# Autodesk Inventor assembly: bett_V3_teil3_klappe
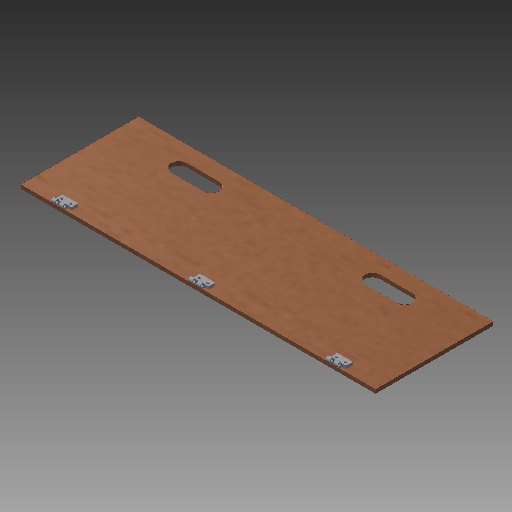
[picture p0: Inventor's stored thumbnail of the model, 512x512]
Saved by Autodesk Inventor 2018 (Build 220112000, 112)
## iProperties
Created: 2020-03-29
Part Number: bett_V3_teil3_klappe
Material: Generisch
Document SubType Name: Assembly
Designer: wepet
Mass: 2.61491 g
Surface Area: 84.4948 cm^2
Volume: 4.7078 cm^3
Density: 0.555441 g/cm^3
Author: wepet
## Documents named in this file (4)
- C:\Users\wepet\Downloads\anhaenger\current\details\bett\bett_V3\bett_V3_teil3_klappe.iam
- C:\Users\wepet\Downloads\anhaenger\current\details\bett\bett_V3\bett_V3_detail_deckplatte_klappe.ipt
- C:\Users\wepet\Downloads\anhaenger\current\details\bett\details\item_scharnier_1_teil.ipt
- C:\Users\wepet\Downloads\anhaenger\current\details\bett\details\item_scharnier_2_teil.ipt
## Components (6 placed, 3 different names)
1. bett_V3_detail_deckplatte_klappe:1 — Passend:1, Passend:2, Passend:3, Passend:4, Passend:5, Passend:6, Fluchtend:1, Fluchtend:2, Fluchtend:3, Passend:7, Passend:8, Passend:9, Passend:10, Fluchtend:4, Fluchtend:5, Passend:11, Fluchtend:6, Passend:12
2. item_scharnier_1_teil:1 — Passend:7, Passend:10, Fluchtend:4
3. item_scharnier_1_teil:2 — Passend:8, Passend:9, Fluchtend:5
4. item_scharnier_2_teil:1 — Passend:2, Passend:6, Fluchtend:1
5. item_scharnier_2_teil:2 — Passend:1, Passend:5, Fluchtend:3
6. item_scharnier_2_teil:3 — Passend:3, Passend:4, Fluchtend:2
## Relationships (18: Mate 12, Flush 6)
- Passend:1 [Mate]: bett_V3_detail_deckplatte_klappe:1 ↔ item_scharnier_2_teil:2
- Passend:2 [Mate]: bett_V3_detail_deckplatte_klappe:1 ↔ item_scharnier_2_teil:1
- Passend:3 [Mate]: bett_V3_detail_deckplatte_klappe:1 ↔ item_scharnier_2_teil:3
- Passend:4 [Mate] (-2.9 mm): bett_V3_detail_deckplatte_klappe:1 ↔ item_scharnier_2_teil:3
- Passend:5 [Mate] (-2.9 mm): bett_V3_detail_deckplatte_klappe:1 ↔ item_scharnier_2_teil:2
- Passend:6 [Mate] (-2.9 mm): bett_V3_detail_deckplatte_klappe:1 ↔ item_scharnier_2_teil:1
- Fluchtend:1 [Flush] (10 mm): bett_V3_detail_deckplatte_klappe:1 ↔ item_scharnier_2_teil:1
- Fluchtend:2 [Flush] (10 mm): bett_V3_detail_deckplatte_klappe:1 ↔ item_scharnier_2_teil:3
- Fluchtend:3 [Flush] (52.6 mm): bett_V3_detail_deckplatte_klappe:1 ↔ item_scharnier_2_teil:2
- Passend:7 [Mate]: bett_V3_detail_deckplatte_klappe:1 ↔ item_scharnier_1_teil:1
- Passend:8 [Mate]: bett_V3_detail_deckplatte_klappe:1 ↔ item_scharnier_1_teil:2
- Passend:9 [Mate] (-6.9 mm): bett_V3_detail_deckplatte_klappe:1 ↔ item_scharnier_1_teil:2
- Passend:10 [Mate] (-6.9 mm): bett_V3_detail_deckplatte_klappe:1 ↔ item_scharnier_1_teil:1
- Fluchtend:4 [Flush] (3 mm): bett_V3_detail_deckplatte_klappe:1 ↔ item_scharnier_1_teil:1
- Fluchtend:5 [Flush] (3 mm): bett_V3_detail_deckplatte_klappe:1 ↔ item_scharnier_1_teil:2
- Passend:11 [Mate]: bett_V3_detail_deckplatte_klappe:1
- Fluchtend:6 [Flush]: bett_V3_detail_deckplatte_klappe:1
- Passend:12 [Mate]: bett_V3_detail_deckplatte_klappe:1
